# Autodesk Inventor assembly: Chuck Assembly
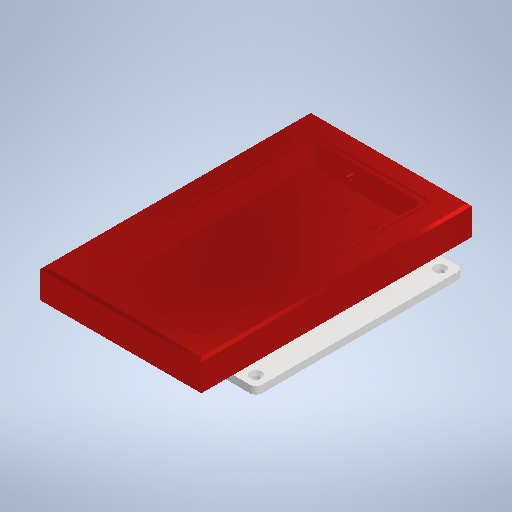
[picture p0: Inventor's stored thumbnail of the model, 512x512]
Saved by Autodesk Inventor 2025 (Build 290162000, 162)
## iProperties
Created: 2024-10-23
Part Number: Chuck Assembly
Document SubType Name: Assembly
Designer: Caleb Fangmeier
Author: Caleb Fangmeier
## Documents named in this file (3)
- C:\Users\cfang\Desktop\nebraska-silicon-lab\Hardware\Wirebonder\BU\Chuck Assembly.iam
- C:\Users\cfang\Desktop\nebraska-silicon-lab\Hardware\Wirebonder\BU\Chuck Adapter Plate.ipt
- C:\Users\cfang\Desktop\nebraska-silicon-lab\Hardware\ETL\Module Assembly\Chuck - V3\Chuck - V3.ipt
## Components (2 placed, 2 different names)
1. Chuck Adapter Plate:1 — Mate:1, Insert:1, Insert:2
2. Chuck - V3:1 — Mate:1, Insert:1, Insert:2
## Relationships (3: Insert 2, Mate 1)
- Mate:1: Chuck Adapter Plate:1 ↔ Chuck - V3:1
- Insert:1: Chuck Adapter Plate:1 ↔ Chuck - V3:1
- Insert:2: Chuck Adapter Plate:1 ↔ Chuck - V3:1
